# Autodesk Inventor assembly: Rubik's Cube Solver
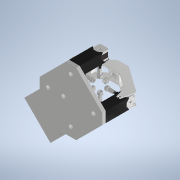
[picture p0: Inventor's stored thumbnail of the model, 180x180]
Saved by Autodesk Inventor 2021 (Build 250183000, 183)
## iProperties
Created: 2021-06-02
Part Number: Rubik's Cube Solver
Document SubType Name: Assembly
Designer: Marc
Author: Marc
## Documents named in this file (9)
- C:\Users\Marc\Documents\Projectes\Rubik's Cube Solver\Prototip Definitiu\Rubik's Cube Solver.iam
- C:\Users\Marc\Documents\Projectes\Rubik's Cube Solver\Prototip Definitiu\Components\Base.ipt
- C:\Users\Marc\Documents\Projectes\Rubik's Cube Solver\Prototip Definitiu\Torre Pont+Motor.iam
- C:\Users\Marc\Documents\Projectes\Rubik's Cube Solver\Prototip Definitiu\Torre+Motor.iam
- C:\Users\Marc\Documents\Projectes\Rubik's Cube Solver\Prototip Definitiu\Pont+Motor.iam
- C:\Users\Marc\Documents\Projectes\Rubik's Cube Solver\Prototip Definitiu\Components\Suport_Cam.ipt
- C:\Users\Marc\Documents\Projectes\Rubik's Cube Solver\Prototip Definitiu\Components\LifeCamSubj.ipt
- C:\Users\Marc\Documents\Projectes\Rubik's Cube Solver\Prototip Definitiu\Components\Subj_Cube.ipt
- C:\Users\Marc\Documents\Projectes\Rubik's Cube Solver\Prototip Definitiu\Torre Inferior+Motor+Eix.iam
## Components (10 placed, 8 different names)
1. Base:1 — Coincidencia:1, Nivelación:1, Nivelación:2, Coincidencia:2, Nivelación:3, Nivelación:4, Coincidencia:3, Nivelación:5, Coincidencia:4, Coincidencia:5, Nivelación:6, Coincidencia:6, Coincidencia:9, Nivelación:7, Ángulo:1, Coincidencia:12, Nivelación:8, Nivelación:9, Coincidencia:13, Coincidencia:14
2. Torre Pont+Motor:1 [sub-assembly] — Coincidencia:1, Nivelación:1, Nivelación:2, Coincidencia:7, Coincidencia:8
3. Torre Pont+Motor:2 [sub-assembly] — Coincidencia:2, Nivelación:3, Nivelación:4
4. Torre+Motor:1 [sub-assembly] — Coincidencia:5, Nivelación:6, Coincidencia:6
5. Torre+Motor:2 [sub-assembly] — Coincidencia:3, Nivelación:5, Coincidencia:4
6. Pont+Motor:1 [sub-assembly] — Coincidencia:7, Coincidencia:8
7. Suport_Cam:1 — Coincidencia:9, Nivelación:7, Ángulo:1, Coincidencia:10, Coincidencia:11
8. LifeCamSubj:1 — Coincidencia:10, Coincidencia:11
9. Subj_Cube:1 — Coincidencia:12, Nivelación:8, Nivelación:9
10. Torre Inferior+Motor+Eix:1 [sub-assembly] — Coincidencia:13, Coincidencia:14
## Relationships (24: Mate 14, Flush 9, Angle 1)
- Coincidencia:1 [Mate]: Base:1 ↔ Torre Pont+Motor:1
- Nivelación:1 [Flush]: Base:1 ↔ Torre Pont+Motor:1
- Nivelación:2 [Flush] (120.75 mm): Base:1 ↔ Torre Pont+Motor:1
- Coincidencia:2 [Mate]: Base:1 ↔ Torre Pont+Motor:2
- Nivelación:3 [Flush]: Base:1 ↔ Torre Pont+Motor:2
- Nivelación:4 [Flush] (120.75 mm): Base:1 ↔ Torre Pont+Motor:2
- Coincidencia:3 [Mate]: Base:1 ↔ Torre+Motor:2
- Nivelación:5 [Flush]: Base:1 ↔ Torre+Motor:2
- Coincidencia:4 [Mate]: Base:1 ↔ Torre+Motor:2
- Coincidencia:5 [Mate]: Base:1 ↔ Torre+Motor:1
- Nivelación:6 [Flush]: Base:1 ↔ Torre+Motor:1
- Coincidencia:6 [Mate]: Base:1 ↔ Torre+Motor:1
- Coincidencia:7 [Mate]: Torre Pont+Motor:1 ↔ Pont+Motor:1
- Coincidencia:8 [Mate] (0.5 mm): Torre Pont+Motor:1 ↔ Pont+Motor:1
- Coincidencia:9 [Mate]: Base:1 ↔ Suport_Cam:1
- Nivelación:7 [Flush]: Base:1 ↔ Suport_Cam:1
- Ángulo:1 [Angle] (90 deg): Base:1 ↔ Suport_Cam:1
- Coincidencia:10 [Mate]: Suport_Cam:1 ↔ LifeCamSubj:1
- Coincidencia:11 [Mate]: Suport_Cam:1 ↔ LifeCamSubj:1
- Coincidencia:12 [Mate]: Base:1 ↔ Subj_Cube:1
- Nivelación:8 [Flush]: Base:1 ↔ Subj_Cube:1
- Nivelación:9 [Flush] (35 mm): Base:1 ↔ Subj_Cube:1
- Coincidencia:13 [Mate]: Base:1 ↔ Torre Inferior+Motor+Eix:1
- Coincidencia:14 [Mate]: Base:1 ↔ Torre Inferior+Motor+Eix:1
